# Autodesk Inventor assembly: CHASSIS
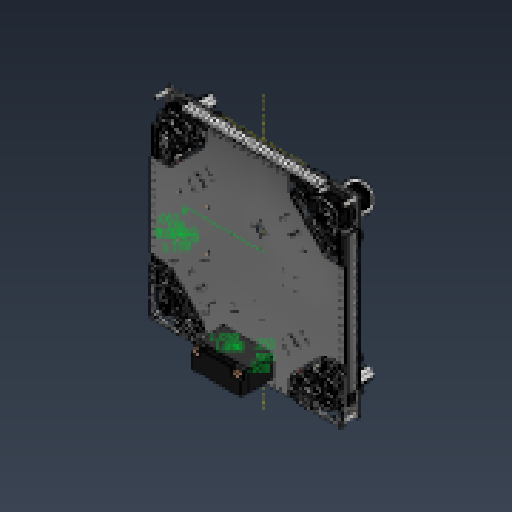
[picture p0: Inventor's stored thumbnail of the model, 512x512]
Saved by Autodesk Inventor 2026 (Build 300175050, 175E)
## iProperties
Created: 2026-01-19
Part Number: CHASSIS
Document SubType Name: Assembly
Designer: Jthib
Mass: 23715 g
Surface Area: 48188 cm^2
Volume: 9124.95 cm^3
Density: 2.59892 g/cm^3
Author: Jthib
## Documents named in this file (16)
- C:\Users\Jthib\Documents\GitHub\2026-Robot-Mechanical\Chassis\CHASSIS.iam
- C:\Users\Jthib\Documents\GitHub\2026-Robot-Mechanical\#1_CAD Library\SDS MK4i Swerve\ASSY,MK4i,HIGH,Swerve_Module.iam
- C:\Users\Jthib\Documents\GitHub\2026-Robot-Mechanical\Chassis\FRAME,MAXTUBE.ipt
- C:\Users\Jthib\Documents\GitHub\2026-Robot-Mechanical\#1_CAD Library\SDS MK4i Swerve\SDS Colson Wheel Kit.ipt
- C:\Users\Jthib\Documents\GitHub\2026-Robot-Mechanical\Chassis\PLATE,BELLYPAN.ipt
- C:\Users\Jthib\Documents\GitHub\2026-Robot-Mechanical\Chassis\PLATE,MOUNT,ELECTRONICS.ipt
- C:\Users\Jthib\Documents\GitHub\2026-Robot-Mechanical\#1_CAD Library\Motors\MOTOR,REV,NEO,V1-1.ipt
- C:\Users\Jthib\Documents\GitHub\2026-Robot-Mechanical\Chassis\PLATE,CLAMP,MK4i,Swerve,CUSTOM.ipt
- C:\Users\Jthib\Documents\GitHub\2026-Robot-Mechanical\#1_CAD Library\Electronics\CONTROLS,PDH.ipt
- C:\Users\Jthib\Documents\GitHub\2026-Robot-Mechanical\#1_CAD Library\Electronics\CONTROLS,ROBO_RIO.ipt
- C:\Users\Jthib\Documents\GitHub\2026-Robot-Mechanical\#1_CAD Library\Electronics\CONTROLS,SPARK_MAX.ipt
- C:\Users\Jthib\Documents\GitHub\2026-Robot-Mechanical\#1_CAD Library\Electronics\CONTROLS,VRM.ipt
- C:\Users\Jthib\Documents\GitHub\2026-Robot-Mechanical\#1_CAD Library\Electronics\BATTERY,12V.ipt
- C:\Users\Jthib\Documents\GitHub\2026-Robot-Mechanical\Shooter\Shooter - Front Motors\3DPRINT,SPARK_MAX,MOUNT.ipt
- C:\Users\Jthib\Documents\GitHub\2026-Robot-Mechanical\Chassis\PLATE,MOUNT,BATTERY.ipt
- C:\Users\Jthib\Documents\GitHub\2026-Robot-Mechanical\Chassis\MOUNT,FLANGE,BELLYPAN.ipt
## Components (53 placed, 15 different names)
1. ASSY,MK4i,HIGH,Swerve_Module:1 [sub-assembly] — Mate:1, Mate:4, Insert:1, Insert:5, Insert:6, Insert:7, Insert:8, Mate:26, Mate:43, Mate:48, Mate:50
2. ASSY,MK4i,HIGH,Swerve_Module:2 [sub-assembly] — Mate:5, Mate:24, Insert:2, Insert:9, Insert:10, Insert:11, Insert:12
3. ASSY,MK4i,HIGH,Swerve_Module:3 [sub-assembly] — Mate:16, Mate:20, Insert:3, Flush:1, Flush:2, Insert:13, Insert:14, Insert:15, Insert:16
4. ASSY,MK4i,HIGH,Swerve_Module:4 [sub-assembly] — Mate:13, Insert:4, Insert:17, Insert:18, Insert:19, Insert:20
5. FRAME,MAXTUBE:1 — Mate:1, Mate:5, Symmetry:2, Mate:29, Mate:35, Flush:35, Mate:60, Mate:61, Insert:27, Insert:28, Insert:29, Insert:30
6. FRAME,MAXTUBE:2 — Mate:20, Symmetry:1, Mate:30, Mate:31, Flush:36, Mate:62, Mate:63, Insert:21, Insert:22
7. FRAME,MAXTUBE:3 — Mate:13, Mate:16, Mate:25, Flush:3, Symmetry:2, Insert:31, Insert:32, Insert:33, Insert:34
8. FRAME,MAXTUBE:4 — Mate:4, Flush:4, Symmetry:1, Mate:27, Mate:28, Flush:34, Insert:23, Insert:24, Insert:25, Insert:26
9. SDS Colson Wheel Kit:1 — Insert:2
10. SDS Colson Wheel Kit:2 — Insert:3
11. SDS Colson Wheel Kit:3 — Insert:4
12. SDS Colson Wheel Kit:4 — Insert:1
13. PLATE,BELLYPAN:1 — Flush:1, Flush:2, Mate:35
14. PLATE,MOUNT,ELECTRONICS:1 — Mate:25, Flush:3, Flush:4, Mate:36, Mate:37, Mate:38, Mate:39, Mate:47, Mate:52, Mate:53, Mate:54, Mate:55, Mate:56, Mate:57, Mate:58, Mate:59
15. MOTOR,REV,NEO,V1-1:1 — Insert:5, Insert:6
16. MOTOR,REV,NEO,V1-1:2 — Insert:7, Insert:8
17. MOTOR,REV,NEO,V1-1:3 — Insert:9, Insert:10
18. MOTOR,REV,NEO,V1-1:4 — Insert:11, Insert:12
19. MOTOR,REV,NEO,V1-1:5 — Insert:13, Insert:14
20. MOTOR,REV,NEO,V1-1:6 — Insert:15, Insert:16
21. MOTOR,REV,NEO,V1-1:7 — Insert:17, Insert:18
22. MOTOR,REV,NEO,V1-1:8 — Insert:19, Insert:20
23. PLATE,CLAMP,MK4i,Swerve,CUSTOM:1 — Mate:26, Mate:27, Mate:28
24. PLATE,CLAMP,MK4i,Swerve,CUSTOM:2 — Mate:29, Mate:30, Mate:31
25. CONTROLS,PDH:1 — Mate:37, Mate:52, Mate:53
26. CONTROLS,ROBO_RIO:1 — Mate:36, Mate:56, Mate:57
27. CONTROLS,VRM:1 — Mate:38, Mate:54, Mate:55
28. BATTERY,12V:1 — Flush:34, Mate:58, Mate:59
29. PLATE,MOUNT,BATTERY:1 — Flush:35, Mate:60, Mate:61
30. MOUNT,FLANGE,BELLYPAN:1 — Flush:36, Mate:62, Mate:63
31. MOUNT,FLANGE,BELLYPAN:2 — Insert:21, Insert:22
32. MOUNT,FLANGE,BELLYPAN:3 — Insert:23, Insert:24
33. MOUNT,FLANGE,BELLYPAN:4 — Insert:25, Insert:26
34. MOUNT,FLANGE,BELLYPAN:5 — Insert:27, Insert:28
35. MOUNT,FLANGE,BELLYPAN:6 — Insert:29, Insert:30
36. MOUNT,FLANGE,BELLYPAN:7 — Insert:31, Insert:32
37. MOUNT,FLANGE,BELLYPAN:8 — Insert:33, Insert:34
38. CONTROLS,SPARK_MAX:1 — Mate:39, Mate:43, Mate:49, Mate:50
39. 3DPRINT,SPARK_MAX,MOUNT:1
40. CONTROLS,SPARK_MAX:2 — Mate:47, Mate:48, Mate:49
41. 3DPRINT,SPARK_MAX,MOUNT:2
42. CONTROLS,SPARK_MAX:3
43. 3DPRINT,SPARK_MAX,MOUNT:3
44. CONTROLS,SPARK_MAX:4
45. 3DPRINT,SPARK_MAX,MOUNT:4
46. CONTROLS,SPARK_MAX:5
47. 3DPRINT,SPARK_MAX,MOUNT:5
48. CONTROLS,SPARK_MAX:6
49. 3DPRINT,SPARK_MAX,MOUNT:6
50. CONTROLS,SPARK_MAX:7
51. 3DPRINT,SPARK_MAX,MOUNT:7
52. CONTROLS,SPARK_MAX:8
53. 3DPRINT,SPARK_MAX,MOUNT:8
## Component patterns: (4 elements, first: CONTROLS,SPARK_MAX:1 + 3DPRINT,SPARK_MAX,MOUNT:1 + CONTROLS,SPARK_MAX:2 + 3DPRINT,SPARK_MAX,MOUNT:2)
## Relationships (85: Mate 42, Insert 34, Flush 7, Symmetry 2)
- Mate:1: ASSY,MK4i,HIGH,Swerve_Module:1 ↔ FRAME,MAXTUBE:1
- Mate:4: ASSY,MK4i,HIGH,Swerve_Module:1 ↔ FRAME,MAXTUBE:4
- Mate:5: ASSY,MK4i,HIGH,Swerve_Module:2 ↔ FRAME,MAXTUBE:1
- Mate:13: ASSY,MK4i,HIGH,Swerve_Module:4 ↔ FRAME,MAXTUBE:3
- Mate:16: ASSY,MK4i,HIGH,Swerve_Module:3 ↔ FRAME,MAXTUBE:3
- Mate:20: ASSY,MK4i,HIGH,Swerve_Module:3 ↔ FRAME,MAXTUBE:2
- Mate:24 (95.25 mm): ASSY,MK4i,HIGH,Swerve_Module:2
- Insert:1: ASSY,MK4i,HIGH,Swerve_Module:1 ↔ SDS Colson Wheel Kit:4
- Insert:2: ASSY,MK4i,HIGH,Swerve_Module:2 ↔ SDS Colson Wheel Kit:1
- Insert:3: ASSY,MK4i,HIGH,Swerve_Module:3 ↔ SDS Colson Wheel Kit:2
- Insert:4: ASSY,MK4i,HIGH,Swerve_Module:4 ↔ SDS Colson Wheel Kit:3
- Flush:1: ASSY,MK4i,HIGH,Swerve_Module:3 ↔ PLATE,BELLYPAN:1
- Flush:2: ASSY,MK4i,HIGH,Swerve_Module:3 ↔ PLATE,BELLYPAN:1
- Mate:25: FRAME,MAXTUBE:3 ↔ PLATE,MOUNT,ELECTRONICS:1
- Flush:3: FRAME,MAXTUBE:3 ↔ PLATE,MOUNT,ELECTRONICS:1
- Flush:4: FRAME,MAXTUBE:4 ↔ PLATE,MOUNT,ELECTRONICS:1
- Symmetry:1: FRAME,MAXTUBE:2 ↔ FRAME,MAXTUBE:4
- Symmetry:2: FRAME,MAXTUBE:1 ↔ FRAME,MAXTUBE:3
- Insert:5: ASSY,MK4i,HIGH,Swerve_Module:1 ↔ MOTOR,REV,NEO,V1-1:1
- Insert:6: ASSY,MK4i,HIGH,Swerve_Module:1 ↔ MOTOR,REV,NEO,V1-1:1
- Insert:7: ASSY,MK4i,HIGH,Swerve_Module:1 ↔ MOTOR,REV,NEO,V1-1:2
- Insert:8: ASSY,MK4i,HIGH,Swerve_Module:1 ↔ MOTOR,REV,NEO,V1-1:2
- Insert:9: ASSY,MK4i,HIGH,Swerve_Module:2 ↔ MOTOR,REV,NEO,V1-1:3
- Insert:10: ASSY,MK4i,HIGH,Swerve_Module:2 ↔ MOTOR,REV,NEO,V1-1:3
- Insert:11: ASSY,MK4i,HIGH,Swerve_Module:2 ↔ MOTOR,REV,NEO,V1-1:4
- Insert:12: ASSY,MK4i,HIGH,Swerve_Module:2 ↔ MOTOR,REV,NEO,V1-1:4
- Insert:13: ASSY,MK4i,HIGH,Swerve_Module:3 ↔ MOTOR,REV,NEO,V1-1:5
- Insert:14: ASSY,MK4i,HIGH,Swerve_Module:3 ↔ MOTOR,REV,NEO,V1-1:5
- Insert:15: ASSY,MK4i,HIGH,Swerve_Module:3 ↔ MOTOR,REV,NEO,V1-1:6
- Insert:16: ASSY,MK4i,HIGH,Swerve_Module:3 ↔ MOTOR,REV,NEO,V1-1:6
- Insert:17: ASSY,MK4i,HIGH,Swerve_Module:4 ↔ MOTOR,REV,NEO,V1-1:7
- Insert:18: ASSY,MK4i,HIGH,Swerve_Module:4 ↔ MOTOR,REV,NEO,V1-1:7
- Insert:19: ASSY,MK4i,HIGH,Swerve_Module:4 ↔ MOTOR,REV,NEO,V1-1:8
- Insert:20: ASSY,MK4i,HIGH,Swerve_Module:4 ↔ MOTOR,REV,NEO,V1-1:8
- Mate:26: ASSY,MK4i,HIGH,Swerve_Module:1 ↔ PLATE,CLAMP,MK4i,Swerve,CUSTOM:1
- Mate:27: FRAME,MAXTUBE:4 ↔ PLATE,CLAMP,MK4i,Swerve,CUSTOM:1
- Mate:28: FRAME,MAXTUBE:4 ↔ PLATE,CLAMP,MK4i,Swerve,CUSTOM:1
- Mate:29: FRAME,MAXTUBE:1 ↔ PLATE,CLAMP,MK4i,Swerve,CUSTOM:2
- Mate:30: FRAME,MAXTUBE:2 ↔ PLATE,CLAMP,MK4i,Swerve,CUSTOM:2
- Mate:31: FRAME,MAXTUBE:2 ↔ PLATE,CLAMP,MK4i,Swerve,CUSTOM:2
- Flush:34: FRAME,MAXTUBE:4 ↔ BATTERY,12V:1
- Mate:35: FRAME,MAXTUBE:1 ↔ PLATE,BELLYPAN:1
- Mate:36: PLATE,MOUNT,ELECTRONICS:1 ↔ CONTROLS,ROBO_RIO:1
- Mate:37: PLATE,MOUNT,ELECTRONICS:1 ↔ CONTROLS,PDH:1
- Mate:38: PLATE,MOUNT,ELECTRONICS:1 ↔ CONTROLS,VRM:1
- Mate:39: PLATE,MOUNT,ELECTRONICS:1 ↔ CONTROLS,SPARK_MAX:1
- [Mate]: CONTROLS,SPARK_MAX:1 ↔ 3DPRINT,SPARK_MAX,MOUNT:1
- [Mate]: CONTROLS,SPARK_MAX:1 ↔ 3DPRINT,SPARK_MAX,MOUNT:1
- [Mate]: CONTROLS,SPARK_MAX:1 ↔ 3DPRINT,SPARK_MAX,MOUNT:1
- Mate:43 (38.1 mm): ASSY,MK4i,HIGH,Swerve_Module:1 ↔ CONTROLS,SPARK_MAX:1
- [Mate]: CONTROLS,SPARK_MAX:2 ↔ 3DPRINT,SPARK_MAX,MOUNT:2
- [Mate]: CONTROLS,SPARK_MAX:2 ↔ 3DPRINT,SPARK_MAX,MOUNT:2
- [Mate]: CONTROLS,SPARK_MAX:2 ↔ 3DPRINT,SPARK_MAX,MOUNT:2
- Mate:47: PLATE,MOUNT,ELECTRONICS:1 ↔ CONTROLS,SPARK_MAX:2
- Mate:48 (38.1 mm): ASSY,MK4i,HIGH,Swerve_Module:1 ↔ CONTROLS,SPARK_MAX:2
- Mate:49 (15.875 mm): CONTROLS,SPARK_MAX:1 ↔ CONTROLS,SPARK_MAX:2
- Mate:50 (7.9375 mm): ASSY,MK4i,HIGH,Swerve_Module:1 ↔ CONTROLS,SPARK_MAX:1
- Mate:52: PLATE,MOUNT,ELECTRONICS:1 ↔ CONTROLS,PDH:1
- Mate:53: PLATE,MOUNT,ELECTRONICS:1 ↔ CONTROLS,PDH:1
- Mate:54: PLATE,MOUNT,ELECTRONICS:1 ↔ CONTROLS,VRM:1
- Mate:55: PLATE,MOUNT,ELECTRONICS:1 ↔ CONTROLS,VRM:1
- Mate:56: PLATE,MOUNT,ELECTRONICS:1 ↔ CONTROLS,ROBO_RIO:1
- Mate:57: PLATE,MOUNT,ELECTRONICS:1 ↔ CONTROLS,ROBO_RIO:1
- Mate:58: PLATE,MOUNT,ELECTRONICS:1 ↔ BATTERY,12V:1
- Mate:59 (3.4925 mm): PLATE,MOUNT,ELECTRONICS:1 ↔ BATTERY,12V:1
- Flush:35: FRAME,MAXTUBE:1 ↔ PLATE,MOUNT,BATTERY:1
- Mate:60: FRAME,MAXTUBE:1 ↔ PLATE,MOUNT,BATTERY:1
- Mate:61: FRAME,MAXTUBE:1 ↔ PLATE,MOUNT,BATTERY:1
- Flush:36: FRAME,MAXTUBE:2 ↔ MOUNT,FLANGE,BELLYPAN:1
- Mate:62: FRAME,MAXTUBE:2 ↔ MOUNT,FLANGE,BELLYPAN:1
- Mate:63: FRAME,MAXTUBE:2 ↔ MOUNT,FLANGE,BELLYPAN:1
- Insert:21: FRAME,MAXTUBE:2 ↔ MOUNT,FLANGE,BELLYPAN:2
- Insert:22: FRAME,MAXTUBE:2 ↔ MOUNT,FLANGE,BELLYPAN:2
- Insert:23: FRAME,MAXTUBE:4 ↔ MOUNT,FLANGE,BELLYPAN:3
- Insert:24: FRAME,MAXTUBE:4 ↔ MOUNT,FLANGE,BELLYPAN:3
- Insert:25: FRAME,MAXTUBE:4 ↔ MOUNT,FLANGE,BELLYPAN:4
- Insert:26: FRAME,MAXTUBE:4 ↔ MOUNT,FLANGE,BELLYPAN:4
- Insert:27: FRAME,MAXTUBE:1 ↔ MOUNT,FLANGE,BELLYPAN:5
- Insert:28: FRAME,MAXTUBE:1 ↔ MOUNT,FLANGE,BELLYPAN:5
- Insert:29: FRAME,MAXTUBE:1 ↔ MOUNT,FLANGE,BELLYPAN:6
- Insert:30: FRAME,MAXTUBE:1 ↔ MOUNT,FLANGE,BELLYPAN:6
- Insert:31: FRAME,MAXTUBE:3 ↔ MOUNT,FLANGE,BELLYPAN:7
- Insert:32: FRAME,MAXTUBE:3 ↔ MOUNT,FLANGE,BELLYPAN:7
- Insert:33: FRAME,MAXTUBE:3 ↔ MOUNT,FLANGE,BELLYPAN:8
- Insert:34: FRAME,MAXTUBE:3 ↔ MOUNT,FLANGE,BELLYPAN:8
## Named parameters: d77_d91 = 0 mm, d78_d94 = 0 mm, d79_d95 = 0 mm
